# Autodesk Inventor assembly: Chain3
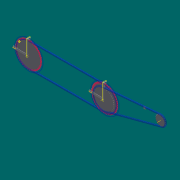
[picture p0: Inventor's stored thumbnail of the model, 180x180]
Saved by Autodesk Inventor 2016 (Build 200138000, 138)
## iProperties
Created: 2017-01-14
Part Number: Chain3
Document SubType Name: Assembly
Designer: katzchristy
Author: katzchristy
## Documents named in this file (7)
- C:\Users\katzchristy\.babun\cygwin\home\katzchristy\ChainguardV4.0\Chain4.iam
- Chain4.iam
- C:\Users\katzchristy\.babun\cygwin\home\katzchristy\ChainguardV4.0\Chain Drive1.iam
- C:\Users\katzchristy\.babun\cygwin\home\katzchristy\ChainguardV4.0\Chain Drive2.iam
- C:\Users\katzchristy\.babun\cygwin\home\katzchristy\ChainguardV4.0\Ell-Tab.ipt
- C:\Users\katzchristy\.babun\cygwin\home\katzchristy\ChainguardV4.0\Ell-Tab_small.ipt
- C:\Users\katzchristy\.babun\cygwin\home\katzchristy\ChainguardV4.0\fender.ipt
## Components (6 placed, 4 different names)
1. Chain Drive:1 [sub-assembly] — Rotational:1, Mate:1, Mate:2, Mate:3, Mate:4, Mate:5
2. Chain Drive:2 [sub-assembly] — Rotational:1
3. Ell-Tab:1 — Mate:2, Mate:3
4. Ell-Tab:2 — Mate:4, Mate:5, Flush:1, Flush:2
5. Ell-Tab_small:1 — Mate:6, Flush:1, Flush:2
6. fender:1 — Mate:7
## Relationships (10: Mate 7, Flush 2, RevoluteJoint 1)
- Rotational:1 [RevoluteJoint] (5.08 mm): Chain Drive:1 ↔ Chain Drive:2
- Mate:1: Chain Drive:1
- Mate:2 (8.89 mm): Chain Drive:1 ↔ Ell-Tab:1
- Mate:3: Chain Drive:1 ↔ Ell-Tab:1
- Mate:4 (8.89 mm): Chain Drive:1 ↔ Ell-Tab:2
- Mate:5: Chain Drive:1 ↔ Ell-Tab:2
- Mate:6: Ell-Tab_small:1
- Flush:1 (-304.8 mm): Ell-Tab:2 ↔ Ell-Tab_small:1
- Flush:2 (11.1125 mm): Ell-Tab:2 ↔ Ell-Tab_small:1
- Mate:7: fender:1
